# Autodesk Inventor assembly: VersaPlanetary 500 Hex 1 stage
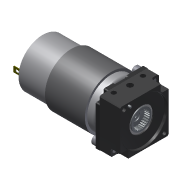
[picture p0: Inventor's stored thumbnail of the model, 180x180]
Saved by Autodesk Inventor 2013 (Build 170138000, 138)
## iProperties
Created: 2013-12-15
Part Number: VersaPlanetary 500 Hex 1 stage
Document SubType Name: Assembly
Designer: Nemo
Author: Nemo
## Documents named in this file (11)
- \\lmss\students\Robotics\CAD Files\COTS Parts\VersaPlanetary\VersaPlanetary RS-775 Input.iam
- \\lmss\students\Robotics\CAD Files\COTS Parts\VersaPlanetary\Components\VersaPlanetary Case Motor Side.ipt
- \\lmss\students\Robotics\CAD Files\COTS Parts\VersaPlanetary\Components\VersaPlanetary Shaft Holder.ipt
- \\lmss\students\Robotics\CAD Files\COTS Parts\Bearings - VexPro\Radial Bearing - 17mm x 26mm x 5mm.ipt
- \\lmss\students\Robotics\CAD Files\COTS Parts\VersaPlanetary\Components\VersaPlanetary RS550 shaft piece.ipt
- \\lmss\students\Robotics\CAD Files\COTS Parts\Fasteners\8-32 SHCS x500.ipt
- \\lmss\students\Robotics\CAD Files\COTS Parts\VersaPlanetary\Components\VersaPlanetary shaft holder clip ring.ipt
- \\lmss\students\Robotics\CAD Files\COTS Parts\VersaPlanetary\Components\VersaPlanetary pin.ipt
- \\lmss\students\Robotics\CAD Files\COTS Parts\VersaPlanetary\Components\VersaPlanetary Mount Plate - RS-775.ipt
- \\lmss\students\Robotics\CAD Files\COTS Parts\Motors\RS775-18V.ipt
- \\lmss\students\Robotics\CAD Files\COTS Parts\Fasteners\M4 SHCS x10.ipt
## Components (12 placed, 10 different names)
1. VersaPlanetary Case Motor Side:1 — Mate:1, Mate:2, Insert:5, Mate:6, Flush:2, Mate:7, Mate:8, Mate:10, Mate:13, Flush:3, Flush:4
2. VersaPlanetary Shaft Holder:1 — Mate:3, Mate:4, Mate:5, Flush:1, Insert:4
3. Radial Bearing - 17mm x 26mm x 5mm:1 — Mate:1, Mate:2, Mate:3, Mate:4
4. VersaPlanetary RS550 shaft piece:1 — Mate:5, Flush:1
5. VersaPlanetary shaft holder clip ring:1 — Insert:4
6. VersaPlanetary pin:1 — Insert:5
7. 8-32 SHCS x500:3 — Mate:10, Mate:11
8. 8-32 SHCS x500:4 — Mate:8, Mate:9
9. VersaPlanetary Mount Plate - RS-775:1 — Mate:6, Flush:2, Mate:7, Mate:9, Mate:11, Insert:6, Insert:7, Insert:8
10. RS775-18V:1 — Insert:8, Mate:12
11. M4 SHCS x10:1 — Insert:6
12. M4 SHCS x10:2 — Insert:7, Mate:12
## Relationships (22: Mate 13, Insert 5, Flush 4)
- Mate:1: VersaPlanetary Case Motor Side:1 ↔ Radial Bearing - 17mm x 26mm x 5mm:1
- Mate:2: VersaPlanetary Case Motor Side:1 ↔ Radial Bearing - 17mm x 26mm x 5mm:1
- Mate:3: VersaPlanetary Shaft Holder:1 ↔ Radial Bearing - 17mm x 26mm x 5mm:1
- Mate:4: VersaPlanetary Shaft Holder:1 ↔ Radial Bearing - 17mm x 26mm x 5mm:1
- Mate:5: VersaPlanetary Shaft Holder:1 ↔ VersaPlanetary RS550 shaft piece:1
- Flush:1: VersaPlanetary Shaft Holder:1 ↔ VersaPlanetary RS550 shaft piece:1
- Insert:4: VersaPlanetary Shaft Holder:1 ↔ VersaPlanetary shaft holder clip ring:1
- Insert:5: VersaPlanetary Case Motor Side:1 ↔ VersaPlanetary pin:1
- Mate:6: VersaPlanetary Case Motor Side:1 ↔ VersaPlanetary Mount Plate - RS-775:1
- Flush:2: VersaPlanetary Case Motor Side:1 ↔ VersaPlanetary Mount Plate - RS-775:1
- Mate:7: VersaPlanetary Case Motor Side:1 ↔ VersaPlanetary Mount Plate - RS-775:1
- Mate:8: VersaPlanetary Case Motor Side:1 ↔ 8-32 SHCS x500:4
- Mate:9: 8-32 SHCS x500:4 ↔ VersaPlanetary Mount Plate - RS-775:1
- Mate:10: VersaPlanetary Case Motor Side:1 ↔ 8-32 SHCS x500:3
- Mate:11: 8-32 SHCS x500:3 ↔ VersaPlanetary Mount Plate - RS-775:1
- Insert:6: VersaPlanetary Mount Plate - RS-775:1 ↔ M4 SHCS x10:1
- Insert:7: VersaPlanetary Mount Plate - RS-775:1 ↔ M4 SHCS x10:2
- Insert:8: VersaPlanetary Mount Plate - RS-775:1 ↔ RS775-18V:1
- Mate:12: RS775-18V:1 ↔ M4 SHCS x10:2
- Mate:13: VersaPlanetary Case Motor Side:1
- Flush:3: VersaPlanetary Case Motor Side:1
- Flush:4: VersaPlanetary Case Motor Side:1
